# Autodesk Inventor assembly: Right_Arm
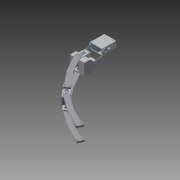
[picture p0: Inventor's stored thumbnail of the model, 180x180]
Saved by Autodesk Inventor 2013 (Build 170138000, 138)
## iProperties
Created: 2014-05-07
Part Number: Right_Arm
Document SubType Name: Assembly
Designer: andou
Mass: 429.088 g
Surface Area: 1516.71 cm^2
Volume: 223.56 cm^3
Density: 1.91934 g/cm^3
Author: andou
## Documents named in this file (16)
- C:\Users\andou\Documents\Inventor\RoboticsProject\project_4\Robot\Arm\Right_Arm\Right_Arm.iam
- C:\Users\andou\Documents\Inventor\RoboticsProject\project_4\Robot\All Common\Serial_Case.ipt
- C:\Users\andou\Documents\Inventor\RoboticsProject\project_4\Robot\Arm\KRS-2542HV.ipt
- C:\Users\andou\Documents\Inventor\RoboticsProject\project_4\Robot\Arm\Horn_Spacer.ipt
- C:\Users\andou\Documents\Inventor\RoboticsProject\project_4\Robot\All Common\Cap(M3-6).ipt
- C:\Users\andou\Documents\Inventor\RoboticsProject\project_4\Robot\All Common\Cap(M4-15).ipt
- C:\Users\andou\Documents\Inventor\RoboticsProject\project_4\Robot\All Common\Nylon_Nat(M4).ipt
- C:\Users\andou\Documents\Inventor\RoboticsProject\project_4\Robot\All Common\Washer(M4).ipt
- C:\Users\andou\Documents\Inventor\RoboticsProject\project_4\Robot\Free_Horn\Free_Horn.iam
- C:\Users\andou\Documents\Inventor\RoboticsProject\project_4\Robot\All Common\Low_Height_Horn.ipt
- C:\Users\andou\Documents\Inventor\RoboticsProject\project_4\Robot\Arm\Arm_Link.ipt
- C:\Users\andou\Documents\Inventor\RoboticsProject\project_4\Robot\Arm\Arm_Link_Shim.ipt
- C:\Users\andou\Documents\Inventor\RoboticsProject\project_4\Robot\Arm\Pitch_Serial_Case.ipt
- C:\Users\andou\Documents\Inventor\RoboticsProject\project_4\Robot\Arm\Yaw_Serial_Case.ipt
- C:\Users\andou\Documents\Inventor\RoboticsProject\project_4\Robot\Arm\Arm_MiniLink.ipt
- C:\Users\andou\Documents\Inventor\RoboticsProject\project_4\Robot\Arm\Arm_MiniLink_Shim.ipt
## Components (40 placed, 15 different names)
1. KRS-2542HV:1 — 挿入:7, 挿入:55, 挿入:56
2. Horn_Spacer:1 — 挿入:8, 挿入:9, 挿入:10, 挿入:35, 挿入:36
3. Cap(M3-6):1 — 挿入:9
4. Cap(M4-15):1 — 挿入:6
5. Nylon_Nat(M4):1 — 挿入:4
6. Washer(M4):1 — 挿入:4, 挿入:86
7. Free_Horn:1 [sub-assembly] — 挿入:6, 挿入:39, 挿入:42
8. Low_Height_Horn:1 — 挿入:7, 挿入:8, 挿入:10
9. KRS-2542HV:2 — 挿入:19, 挿入:70, 挿入:71
10. KRS-2542HV:3 — 挿入:16, 挿入:17, 挿入:20
11. Horn_Spacer:2 — 挿入:22, 挿入:24, 挿入:34, 挿入:72, 挿入:75
12. Horn_Spacer:3 — 挿入:21, 挿入:23, 挿入:33, 挿入:37, 挿入:38
13. Free_Horn:2 [sub-assembly] — 挿入:28, 挿入:68, 挿入:73, 挿入:74
14. Free_Horn:3 [sub-assembly] — 挿入:26, 挿入:27, 挿入:40, 挿入:41
15. Cap(M3-6):2 — 挿入:23
16. Cap(M3-6):3 — 挿入:24
17. Cap(M4-15):2 — 挿入:27
18. Cap(M4-15):4 — 挿入:28
19. Low_Height_Horn:2 — 挿入:20, 挿入:21, 挿入:33
20. Low_Height_Horn:3 — 挿入:19, 挿入:22, 挿入:34
21. Washer(M4):2 — 挿入:29, 挿入:31
22. Washer(M4):3 — 挿入:30, 挿入:69
23. Nylon_Nat(M4):2 — 挿入:29
24. Nylon_Nat(M4):3 — 挿入:30
25. Serial_Case:2 — 挿入:16, 挿入:17, 挿入:26, 挿入:31, 挿入:51, 挿入:52, 挿入:53, 挿入:54
26. Arm_Link:1 — 挿入:35, 挿入:36, 挿入:47, 挿入:49
27. Arm_Link:2 — 挿入:37, 挿入:38, 挿入:43, 挿入:44, メイト:1
28. Arm_Link:3 — 挿入:39, 挿入:42, 挿入:48, 挿入:50
29. Arm_Link:4 — 挿入:40, 挿入:41, 挿入:45, 挿入:46
30. Arm_Link_Shim:1 — 挿入:43, 挿入:44
31. Arm_Link_Shim:2 — 挿入:45, 挿入:46, メイト:1
32. Arm_Link_Shim:3 — 挿入:47, 挿入:49, 挿入:53, 挿入:54
33. Arm_Link_Shim:4 — 挿入:48, 挿入:50, 挿入:51, 挿入:52
34. Pitch_Serial_Case:1 — 挿入:68, 挿入:69, 挿入:70, 挿入:71
35. Yaw_Serial_Case:1 — 挿入:55, 挿入:56, 挿入:76, 挿入:77, 挿入:80, 挿入:83, 挿入:86
36. Arm_MiniLink:1 — 挿入:73, 挿入:74, 挿入:84, 挿入:85
37. Arm_MiniLink:2 — 挿入:72, 挿入:75, 挿入:81, 挿入:82
38. Arm_MiniLink_Shim:1 — 挿入:76, 挿入:80, 挿入:81, 挿入:82
39. Arm_MiniLink_Shim:2 — 挿入:77, 挿入:78, 挿入:79, 挿入:83
40. Arm_MiniLink_Shim:3 — 挿入:78, 挿入:79, 挿入:84, 挿入:85
## Relationships (64: Insert 63, Mate 1)
- 挿入:4 [Insert]: Nylon_Nat(M4):1 ↔ Washer(M4):1
- 挿入:6 [Insert]: Cap(M4-15):1 ↔ Free_Horn:1
- 挿入:7 [Insert]: KRS-2542HV:1 ↔ Low_Height_Horn:1
- 挿入:8 [Insert]: Horn_Spacer:1 ↔ Low_Height_Horn:1
- 挿入:9 [Insert]: Horn_Spacer:1 ↔ Cap(M3-6):1
- 挿入:10 [Insert]: Horn_Spacer:1 ↔ Low_Height_Horn:1
- 挿入:16 [Insert]: KRS-2542HV:3 ↔ Serial_Case:2
- 挿入:17 [Insert]: KRS-2542HV:3 ↔ Serial_Case:2
- 挿入:19 [Insert]: KRS-2542HV:2 ↔ Low_Height_Horn:3
- 挿入:20 [Insert]: KRS-2542HV:3 ↔ Low_Height_Horn:2
- 挿入:21 [Insert]: Horn_Spacer:3 ↔ Low_Height_Horn:2
- 挿入:22 [Insert]: Horn_Spacer:2 ↔ Low_Height_Horn:3
- 挿入:23 [Insert]: Horn_Spacer:3 ↔ Cap(M3-6):2
- 挿入:24 [Insert]: Horn_Spacer:2 ↔ Cap(M3-6):3
- 挿入:26 [Insert]: Free_Horn:3 ↔ Serial_Case:2
- 挿入:27 [Insert]: Free_Horn:3 ↔ Cap(M4-15):2
- 挿入:28 [Insert]: Free_Horn:2 ↔ Cap(M4-15):4
- 挿入:29 [Insert]: Washer(M4):2 ↔ Nylon_Nat(M4):2
- 挿入:30 [Insert]: Washer(M4):3 ↔ Nylon_Nat(M4):3
- 挿入:31 [Insert]: Washer(M4):2 ↔ Serial_Case:2
- 挿入:33 [Insert]: Horn_Spacer:3 ↔ Low_Height_Horn:2
- 挿入:34 [Insert]: Horn_Spacer:2 ↔ Low_Height_Horn:3
- 挿入:35 [Insert]: Horn_Spacer:1 ↔ Arm_Link:1
- 挿入:36 [Insert]: Horn_Spacer:1 ↔ Arm_Link:1
- 挿入:37 [Insert]: Horn_Spacer:3 ↔ Arm_Link:2
- 挿入:38 [Insert]: Horn_Spacer:3 ↔ Arm_Link:2
- 挿入:39 [Insert]: Free_Horn:1 ↔ Arm_Link:3
- 挿入:40 [Insert]: Free_Horn:3 ↔ Arm_Link:4
- 挿入:41 [Insert]: Free_Horn:3 ↔ Arm_Link:4
- 挿入:42 [Insert]: Free_Horn:1 ↔ Arm_Link:3
- 挿入:43 [Insert]: Arm_Link:2 ↔ Arm_Link_Shim:1
- 挿入:44 [Insert]: Arm_Link:2 ↔ Arm_Link_Shim:1
- 挿入:45 [Insert]: Arm_Link:4 ↔ Arm_Link_Shim:2
- 挿入:46 [Insert]: Arm_Link:4 ↔ Arm_Link_Shim:2
- 挿入:47 [Insert]: Arm_Link:1 ↔ Arm_Link_Shim:3
- 挿入:48 [Insert]: Arm_Link:3 ↔ Arm_Link_Shim:4
- 挿入:49 [Insert]: Arm_Link:1 ↔ Arm_Link_Shim:3
- 挿入:50 [Insert]: Arm_Link:3 ↔ Arm_Link_Shim:4
- 挿入:51 [Insert]: Serial_Case:2 ↔ Arm_Link_Shim:4
- 挿入:52 [Insert]: Serial_Case:2 ↔ Arm_Link_Shim:4
- 挿入:53 [Insert]: Serial_Case:2 ↔ Arm_Link_Shim:3
- 挿入:54 [Insert]: Serial_Case:2 ↔ Arm_Link_Shim:3
- 挿入:55 [Insert]: KRS-2542HV:1 ↔ Yaw_Serial_Case:1
- 挿入:56 [Insert]: KRS-2542HV:1 ↔ Yaw_Serial_Case:1
- 挿入:68 [Insert]: Free_Horn:2 ↔ Pitch_Serial_Case:1
- 挿入:69 [Insert]: Washer(M4):3 ↔ Pitch_Serial_Case:1
- 挿入:70 [Insert]: KRS-2542HV:2 ↔ Pitch_Serial_Case:1
- 挿入:71 [Insert]: KRS-2542HV:2 ↔ Pitch_Serial_Case:1
- 挿入:72 [Insert]: Horn_Spacer:2 ↔ Arm_MiniLink:2
- 挿入:73 [Insert]: Free_Horn:2 ↔ Arm_MiniLink:1
- 挿入:74 [Insert]: Free_Horn:2 ↔ Arm_MiniLink:1
- 挿入:75 [Insert]: Horn_Spacer:2 ↔ Arm_MiniLink:2
- メイト:1 [Mate] (1.953 mm): Arm_Link:2 ↔ Arm_Link_Shim:2
- 挿入:76 [Insert]: Yaw_Serial_Case:1 ↔ Arm_MiniLink_Shim:1
- 挿入:77 [Insert]: Yaw_Serial_Case:1 ↔ Arm_MiniLink_Shim:2
- 挿入:78 [Insert]: Arm_MiniLink_Shim:2 ↔ Arm_MiniLink_Shim:3
- 挿入:79 [Insert]: Arm_MiniLink_Shim:2 ↔ Arm_MiniLink_Shim:3
- 挿入:80 [Insert]: Yaw_Serial_Case:1 ↔ Arm_MiniLink_Shim:1
- 挿入:81 [Insert]: Arm_MiniLink:2 ↔ Arm_MiniLink_Shim:1
- 挿入:82 [Insert]: Arm_MiniLink:2 ↔ Arm_MiniLink_Shim:1
- 挿入:83 [Insert]: Yaw_Serial_Case:1 ↔ Arm_MiniLink_Shim:2
- 挿入:84 [Insert]: Arm_MiniLink:1 ↔ Arm_MiniLink_Shim:3
- 挿入:85 [Insert]: Arm_MiniLink:1 ↔ Arm_MiniLink_Shim:3
- 挿入:86 [Insert]: Washer(M4):1 ↔ Yaw_Serial_Case:1
